# Autodesk Inventor assembly: gearhub
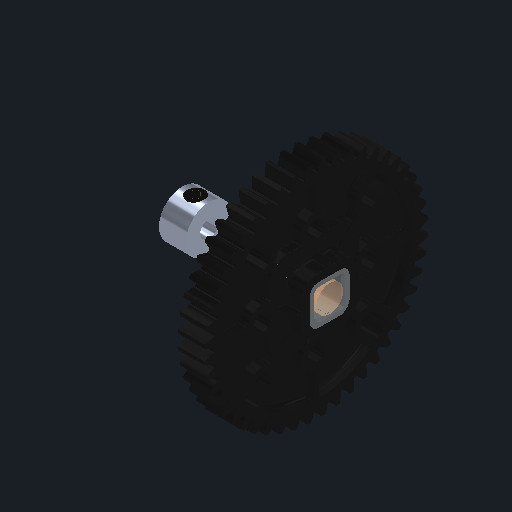
[picture p0: Inventor's stored thumbnail of the model, 512x512]
Saved by Autodesk Inventor 2025 (Build 290162000, 162)
## iProperties
Created: 2024-06-25
Part Number: gearhub
Document SubType Name: Assembly
Designer: Audrey
Author: Audrey
## Documents named in this file (3)
- D:\vex_robotics_high_stakes\hardware\cad\EARLY_SEASON\chassis\drivebay\gearhub.iam
- D:\vex_robotics_high_stakes\hardware\cad\VEX-CAD-Inventor\Motion\Shaft LS\Shaft Collar ipts\Shaft Collar Set Screw.ipt
- D:\vex_robotics_high_stakes\hardware\cad\custom_parts\modified_parts\Half Cut HS 48T Gear, No Insert.ipt
## Components (3 placed, 2 different names)
1. Shaft Collar Set Screw:1 — Insert:1
2. Shaft Collar Set Screw:2 — Insert:1, Insert:2
3. Half Cut HS 48T Gear, No Insert:2 — Insert:2
## Relationships (2: Insert 2)
- Insert:1 (9.525 mm): Shaft Collar Set Screw:1 ↔ Shaft Collar Set Screw:2
- Insert:2: Shaft Collar Set Screw:2 ↔ Half Cut HS 48T Gear, No Insert:2
